# Autodesk Inventor assembly: assembly_enclosure
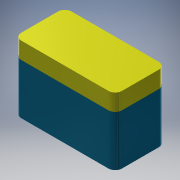
[picture p0: Inventor's stored thumbnail of the model, 180x180]
Saved by Autodesk Inventor 2019 (Build 230136000, 136)
## iProperties
Created: 2019-01-05
Part Number: assembly_enclosure
Document SubType Name: Assembly
Designer: assman
Author: assman
## Documents named in this file (3)
- D:\Inventor\Projects\Tests\enclosure_test\assembly_enclosure.iam
- D:\Inventor\Projects\Tests\enclosure_test\caja.ipt
- D:\Inventor\Projects\Tests\enclosure_test\tapa.ipt
## Components (2 placed, 2 different names)
1. caja:1 — Rigid:1
2. tapa:1 — Rigid:1
## Relationships (1: WeldJoint 1)
- Rigid:1 [WeldJoint]: caja:1 ↔ tapa:1
